# Autodesk Inventor assembly: CaseAnchor
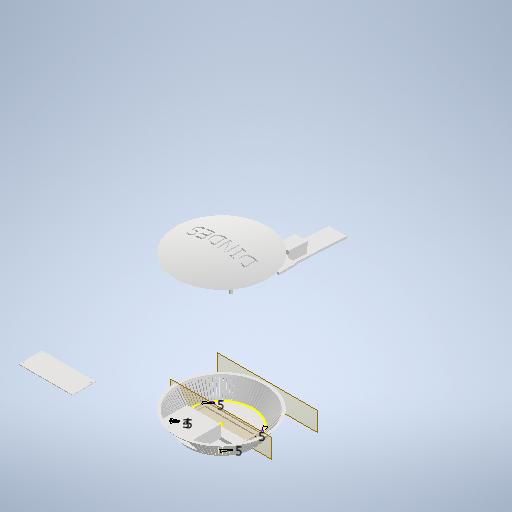
[picture p0: Inventor's stored thumbnail of the model, 512x512]
Saved by Autodesk Inventor 2025.2 (Build 292293000, 293)
## iProperties
Created: 2026-03-13
Part Number: CaseAnchor
Document SubType Name: Assembly
Designer: Periscopio
Author: Periscopio
## Documents named in this file (6)
- C:\Users\Periscopio\Documents\SDV\Polígono\Diseño CAD\Anchor\CaseAnchor.iam
- C:\Users\Periscopio\Documents\SDV\Polígono\Diseño CAD\Anchor\Base.ipt
- C:\Users\Periscopio\Documents\SDV\Polígono\Diseño CAD\Anchor\ESP32_PoE.ipt
- C:\Users\Periscopio\Documents\SDV\Polígono\Diseño CAD\Anchor\PCB.ipt
- C:\Users\Periscopio\Documents\SDV\Polígono\Diseño CAD\Anchor\Tapa.ipt
- C:\Users\Periscopio\Documents\SDV\Polígono\Diseño CAD\Anchor\UWB.ipt
## Components (5 placed, 5 different names)
1. Base:1 — Coincidencia:1
2. ESP32_PoE:1
3. PCB:1 — Coincidencia:1
4. Tapa:1
5. UWB:1
## Relationships (1: Mate 1)
- Coincidencia:1 [Mate]: Base:1 ↔ PCB:1
